# Autodesk Inventor assembly: センサ2個積み右
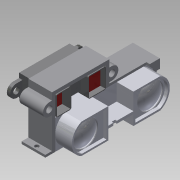
[picture p0: Inventor's stored thumbnail of the model, 180x180]
Saved by Autodesk Inventor 2017 (Build 210142000, 142)
## iProperties
Part Number: センサ2個積み右
Material: 一般
Document SubType Name: Assembly
Designer: HISAAKI
Author: HISAAKI
## Documents named in this file (4)
- C:\Users\HISAAKI\Documents\LYNCS\CanSat\2017種子島\cansat-structure\センサ2個積み右.iam
- C:\Users\HISAAKI\Documents\LYNCS\CanSat\2017種子島\cansat-structure\Sharp_2Y0A710.ipt
- C:\Users\HISAAKI\Documents\LYNCS\CanSat\2017種子島\cansat-structure\SharpDistanceRanger.ipt
- C:\Users\HISAAKI\Documents\LYNCS\CanSat\2017種子島\cansat-structure\センサ冶具.ipt
## Components (3 placed, 3 different names)
1. センサ冶具:1 — メイト:1, メイト:2, メイト:3, メイト:4, メイト:5, メイト:6
2. Sharp_2Y0A710:1 — メイト:1, メイト:2, メイト:3
3. SharpDistanceRanger:1 — メイト:4, メイト:5, メイト:6
## Relationships (6: Mate 6)
- メイト:1 [Mate]: センサ冶具:1 ↔ Sharp_2Y0A710:1
- メイト:2 [Mate]: センサ冶具:1 ↔ Sharp_2Y0A710:1
- メイト:3 [Mate]: センサ冶具:1 ↔ Sharp_2Y0A710:1
- メイト:4 [Mate]: センサ冶具:1 ↔ SharpDistanceRanger:1
- メイト:5 [Mate]: センサ冶具:1 ↔ SharpDistanceRanger:1
- メイト:6 [Mate]: センサ冶具:1 ↔ SharpDistanceRanger:1
